# Autodesk Inventor assembly: compareParts
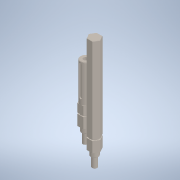
[picture p0: Inventor's stored thumbnail of the model, 180x180]
Saved by Autodesk Inventor 2020.2 (Build 242310000, 310)
## iProperties
Created: 2020-01-26
Part Number: compareParts
Document SubType Name: Assembly
Designer: robst
Author: robst
## Documents named in this file (3)
- C:\git\CAD-Development\robSteele\jeff\compareParts.iam
- C:\git\CAD-Development\robSteele\jeff\am-0153a TB Output Shaft with Magnet.ipt
- C:\git\CAD-Development\robSteele\jeff\am-2566a Short 500 Hex Steel Output Shaft with Magnet for Toughbox Series.iam
## Components (2 placed, 2 different names)
1. am-0153a TB Output Shaft with Magnet:1 — Flush:1, Mate:1
2. am-2566a Short 500 Hex Steel Output Shaft with Magnet for Toughbox Series:1 [sub-assembly] — Flush:1, Mate:1
## Relationships (2: Flush 1, Mate 1)
- Flush:1: am-0153a TB Output Shaft with Magnet:1 ↔ am-2566a Short 500 Hex Steel Output Shaft with Magnet for Toughbox Series:1
- Mate:1 (25.4 mm): am-0153a TB Output Shaft with Magnet:1 ↔ am-2566a Short 500 Hex Steel Output Shaft with Magnet for Toughbox Series:1
